# Autodesk Inventor assembly: Frwing cost
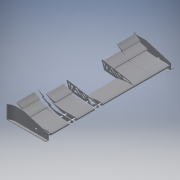
[picture p0: Inventor's stored thumbnail of the model, 180x180]
Saved by Autodesk Inventor 2018.3 (Build 223284000, 284)
## iProperties
Created: 2018-06-13
Part Number: Frwing cost
Material: 一般
Document SubType Name: Assembly
Designer: ku_sk
Author: ku_sk
## Documents named in this file (13)
- D:\ku_sk\ドキュメント\Inventor\Aero\KS-15\コスト用CAD\Frwing\Frwing cost.iam
- D:\ku_sk\ドキュメント\Inventor\Aero\KS-15\コスト用CAD\Frwing\parts\center flap.ipt
- D:\ku_sk\ドキュメント\Inventor\Aero\KS-15\コスト用CAD\Frwing\parts\bracket.ipt
- D:\ku_sk\ドキュメント\Inventor\Aero\KS-15\コスト用CAD\Frwing\parts\main flap.ipt
- D:\ku_sk\ドキュメント\Inventor\Aero\KS-15\コスト用CAD\Frwing\parts\newbracket2.ipt
- D:\ku_sk\ドキュメント\Inventor\Aero\KS-15\コスト用CAD\Frwing\parts\sub flap.ipt
- D:\ku_sk\ドキュメント\Inventor\Aero\KS-15\コスト用CAD\Frwing\parts\newsubflap_top.ipt
- D:\ku_sk\ドキュメント\Inventor\Aero\KS-15\コスト用CAD\Frwing\parts\newsubflap_top1.ipt
- D:\ku_sk\ドキュメント\Inventor\Aero\KS-15\コスト用CAD\Frwing\parts\endplate.ipt
- D:\ku_sk\ドキュメント\Inventor\Aero\KS-15\コスト用CAD\Frwing\parts\endplate1.ipt
- D:\ku_sk\ドキュメント\Inventor\Aero\KS-15\コスト用CAD\Frwing\parts\splitter.iam
- D:\ku_sk\ドキュメント\Inventor\Aero\KS-15\コスト用CAD\Frwing\parts\splitter1.iam
- D:\ku_sk\ドキュメント\Inventor\Aero\KS-15\コスト用CAD\Frwing\parts\core.ipt
## Components (21 placed, 12 different names)
1. center flap:1 — メイト:1, メイト:2, メイト:3, メイト:4, メイト:5, メイト:6, メイト:7, メイト:8, メイト:9, メイト:27
2. bracket:1 — メイト:4, メイト:5, メイト:6, メイト:10, メイト:11, メイト:12, メイト:13
3. bracket:2 — メイト:7, メイト:8, メイト:9, メイト:19, メイト:22, メイト:32
4. main flap:1 — メイト:10, メイト:11, メイト:12, メイト:14, メイト:15, 角度:1
5. main flap:2 — メイト:16, メイト:17, メイト:18, フラッシュ:1, メイト:47, メイト:48, メイト:49, フラッシュ:5
6. main flap:3 — メイト:19, メイト:20, メイト:22, メイト:25, メイト:50
7. main flap:4 — メイト:21, メイト:23, メイト:24, メイト:25, メイト:44, メイト:45, メイト:46
8. newbracket2:1 — メイト:13, メイト:14, メイト:15, メイト:16, メイト:17, メイト:18, メイト:33, メイト:34, メイト:35, メイト:36, メイト:37, メイト:41, メイト:42, メイト:43, フラッシュ:3
9. newbracket2:2 — メイト:20, メイト:21, メイト:23, メイト:24, メイト:26, メイト:27, メイト:28, メイト:29, メイト:30, メイト:31, メイト:38, メイト:39, メイト:40, フラッシュ:2
10. sub flap:1 — メイト:33, メイト:34, メイト:35
11. sub flap:2 — メイト:36, メイト:37, フラッシュ:1
12. sub flap:3 — メイト:30, メイト:31, メイト:32
13. sub flap:4 — メイト:26, メイト:28, メイト:29
14. newsubflap_top:1 — メイト:38, メイト:39, メイト:40
15. newsubflap_top1:1 — メイト:41, メイト:42, メイト:43
16. endplate:1 — メイト:44, メイト:45, メイト:46
17. endplate1:1 — メイト:47, メイト:48, メイト:49, メイト:51, メイト:52
18. splitter:1 [sub-assembly] — メイト:50, フラッシュ:2
19. splitter1:1 [sub-assembly] — フラッシュ:3, 角度:1
20. core:1 — メイト:51, フラッシュ:4
21. core:2 — メイト:52, フラッシュ:4, フラッシュ:5
## Relationships (58: Mate 52, Flush 5, Angle 1)
- メイト:1 [Mate]: center flap:1
- メイト:2 [Mate]: center flap:1
- メイト:3 [Mate]: center flap:1
- メイト:4 [Mate]: center flap:1 ↔ bracket:1
- メイト:5 [Mate]: center flap:1 ↔ bracket:1
- メイト:6 [Mate] (50 mm): center flap:1 ↔ bracket:1
- メイト:7 [Mate]: center flap:1 ↔ bracket:2
- メイト:8 [Mate]: center flap:1 ↔ bracket:2
- メイト:9 [Mate]: center flap:1 ↔ bracket:2
- メイト:10 [Mate]: bracket:1 ↔ main flap:1
- メイト:11 [Mate] (50 mm): bracket:1 ↔ main flap:1
- メイト:12 [Mate]: bracket:1 ↔ main flap:1
- メイト:13 [Mate]: bracket:1 ↔ newbracket2:1
- メイト:14 [Mate] (50 mm): main flap:1 ↔ newbracket2:1
- メイト:15 [Mate]: main flap:1 ↔ newbracket2:1
- メイト:16 [Mate]: main flap:2 ↔ newbracket2:1
- メイト:17 [Mate]: main flap:2 ↔ newbracket2:1
- メイト:18 [Mate] (50 mm): main flap:2 ↔ newbracket2:1
- メイト:19 [Mate]: bracket:2 ↔ main flap:3
- メイト:20 [Mate]: main flap:3 ↔ newbracket2:2
- メイト:21 [Mate]: main flap:4 ↔ newbracket2:2
- メイト:22 [Mate]: bracket:2 ↔ main flap:3
- メイト:23 [Mate]: main flap:4 ↔ newbracket2:2
- メイト:24 [Mate]: main flap:4 ↔ newbracket2:2
- メイト:25 [Mate]: main flap:3 ↔ main flap:4
- メイト:26 [Mate]: newbracket2:2 ↔ sub flap:4
- メイト:27 [Mate]: center flap:1 ↔ newbracket2:2
- メイト:28 [Mate]: newbracket2:2 ↔ sub flap:4
- メイト:29 [Mate]: newbracket2:2 ↔ sub flap:4
- メイト:30 [Mate]: newbracket2:2 ↔ sub flap:3
- メイト:31 [Mate]: newbracket2:2 ↔ sub flap:3
- メイト:32 [Mate]: bracket:2 ↔ sub flap:3
- メイト:33 [Mate]: newbracket2:1 ↔ sub flap:1
- メイト:34 [Mate]: newbracket2:1 ↔ sub flap:1
- メイト:35 [Mate] (50 mm): newbracket2:1 ↔ sub flap:1
- メイト:36 [Mate]: newbracket2:1 ↔ sub flap:2
- メイト:37 [Mate]: newbracket2:1 ↔ sub flap:2
- フラッシュ:1 [Flush]: main flap:2 ↔ sub flap:2
- メイト:38 [Mate]: newbracket2:2 ↔ newsubflap_top:1
- メイト:39 [Mate]: newbracket2:2 ↔ newsubflap_top:1
- メイト:40 [Mate]: newbracket2:2 ↔ newsubflap_top:1
- メイト:41 [Mate]: newbracket2:1 ↔ newsubflap_top1:1
- メイト:42 [Mate] (50 mm): newbracket2:1 ↔ newsubflap_top1:1
- メイト:43 [Mate]: newbracket2:1 ↔ newsubflap_top1:1
- メイト:44 [Mate]: main flap:4 ↔ endplate:1
- メイト:45 [Mate]: main flap:4 ↔ endplate:1
- メイト:46 [Mate]: main flap:4 ↔ endplate:1
- メイト:47 [Mate]: main flap:2 ↔ endplate1:1
- メイト:48 [Mate]: main flap:2 ↔ endplate1:1
- メイト:49 [Mate] (50 mm): main flap:2 ↔ endplate1:1
- メイト:50 [Mate]: main flap:3 ↔ splitter:1
- フラッシュ:2 [Flush]: newbracket2:2 ↔ splitter:1
- フラッシュ:3 [Flush]: newbracket2:1 ↔ splitter1:1
- 角度:1 [Angle] (0 deg): main flap:1 ↔ splitter1:1
- メイト:51 [Mate]: endplate1:1 ↔ core:1
- メイト:52 [Mate]: endplate1:1 ↔ core:2
- フラッシュ:4 [Flush]: core:1 ↔ core:2
- フラッシュ:5 [Flush] (-25 mm): main flap:2 ↔ core:2
